# Autodesk Inventor assembly: 付け根_6_1
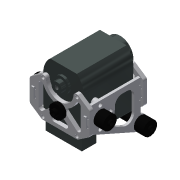
[picture p0: Inventor's stored thumbnail of the model, 180x180]
Saved by Autodesk Inventor 2016 (Build 200138000, 138)
## iProperties
Created: 2016-08-23
Part Number: 付け根_6_1
Material: 一般
Document SubType Name: Assembly
Designer: hiro
Mass: 143.306 g
Surface Area: 289.442 cm^2
Volume: 70.4906 cm^3
Density: 2.03298 g/cm^3
Author: hiro
## Documents named in this file (17)
- C:\Users\haya\Desktop\OpenPlatform\下半身_160823\付け根\付け根_6_1.iam
- C:\Users\haya\Desktop\OpenPlatform\既製品\B3M11xx.ipt
- B3M11xx.ipt
- C:\Users\haya\Desktop\OpenPlatform\下半身_160823\付け根\付け根_メインフレーム_6_1.ipt
- C:\Users\haya\Desktop\OpenPlatform\下半身_160823\付け根\付け根_サブフレーム_6_1.ipt
- C:\Users\haya\Desktop\OpenPlatform\下半身_160823\膝\膝_サブフレーム_6_4.ipt
- C:\Users\haya\Desktop\OpenPlatform\既製品\新規購入\AMP-340E.ipt
- C:\Users\haya\Desktop\OpenPlatform\既製品\新規購入\D3040-7815B.ipt
- C:\Users\haya\Desktop\OpenPlatform\既製品\新規購入\D3040-7115B.ipt
- C:\Users\haya\Desktop\OpenPlatform\既製品\新規購入\BRU-306_5.ipt
- C:\Users\haya\Desktop\OpenPlatform\下半身_160823\追加工\付け根_フリー軸_1_1_ver追加工.ipt
- C:\Users\haya\Desktop\OpenPlatform\既製品\新規購入\LL-7211-10.ipt
- C:\Users\haya\Desktop\OpenPlatform\既製品\新規購入\LL-7211-08.ipt
- C:\Users\haya\Desktop\OpenPlatform\下半身\付け根\付け根_サブフレーム_1_4.ipt
- C:\Users\haya\Desktop\OpenPlatform\既製品\CC-0311-08B.ipt
- C:\Users\haya\Desktop\OpenPlatform\下半身_160823\付け根\付け根_サブフレーム_6_2.ipt
- C:\Users\haya\Desktop\OpenPlatform\既製品\新規購入\BRU-305_5.ipt
## Components (30 placed, 15 different names)
1. B3M11xx:1 — メイト:1, メイト:2, メイト:3, 挿入:9, 挿入:10, 挿入:11, 挿入:12, 挿入:13, 挿入:14, 挿入:15, 挿入:16
2. 付け根_メインフレーム_6_1:1 — 挿入:13, 挿入:14, 挿入:15, 挿入:16, メイト:8, メイト:9, メイト:10, メイト:11, メイト:12, メイト:13, 挿入:60, 挿入:62
3. 付け根_サブフレーム_6_1:1 — メイト:7, メイト:10, メイト:11, メイト:13, 挿入:29, 角度:1, 挿入:31, 挿入:36, 挿入:39, 挿入:40, 挿入:41, 挿入:49
4. 付け根_サブフレーム_6_1:2 — メイト:7, メイト:8, メイト:9, メイト:12, 挿入:30, メイト:14, メイト:15, 挿入:42, 挿入:43, 挿入:44, 挿入:50
5. 付け根_メインフレーム_6_1:2 — 挿入:9, 挿入:10, 挿入:11, 挿入:12, 挿入:58
6. AMP-340E:1 — 挿入:29, 角度:1, 挿入:30
7. D3040-7815B:1 — 挿入:65, 挿入:70
8. D3040-7115B:1 — 挿入:45, 挿入:68
9. BRU-306_5:1 — 挿入:31, 挿入:70
10. BRU-306_5:2 — 挿入:37, 挿入:68
11. 膝_サブフレーム_6_4:1 — メイト:14, メイト:15, 挿入:37
12. 膝_サブフレーム_6_4:2 — 挿入:36
13. 付け根_フリー軸_1_1_ver追加工:1 — 挿入:42, 挿入:43, 挿入:44
14. 付け根_フリー軸_1_1_ver追加工:2 — 挿入:39, 挿入:40, 挿入:41
15. LL-7211-10:1 — 挿入:45
16. LL-7211-08:1 — 挿入:65
17. LL-7211-08:2 — 挿入:54
18. LL-7211-10:2 — 挿入:52
19. D3040-7815B:2 — 挿入:54, 挿入:69
20. D3040-7115B:2 — 挿入:52, 挿入:67
21. BRU-306_5:3 — 挿入:50, 挿入:64, 挿入:67
22. BRU-306_5:4 — 挿入:49, 挿入:66, 挿入:69
23. 膝_サブフレーム_6_4:3 — 挿入:66
24. 膝_サブフレーム_6_4:4 — 挿入:64
25. 付け根_サブフレーム_1_4:1 — 挿入:57
26. CC-0311-08B:1 — 挿入:57, 挿入:58
27. LL-7211-10:3 — 挿入:59
28. D3040-7115B:3 — 挿入:59, 挿入:61, 挿入:63
29. 付け根_サブフレーム_6_2:1 — 挿入:60, 挿入:61
30. BRU-305_5:1 — 挿入:62, 挿入:63
## Relationships (51: Insert 38, Mate 12, Angle 1)
- メイト:1 [Mate] (-19.75 mm): B3M11xx:1
- メイト:2 [Mate] (-25.75 mm): B3M11xx:1
- メイト:3 [Mate] (-16 mm): B3M11xx:1
- メイト:7 [Mate]: 付け根_サブフレーム_6_1:1 ↔ 付け根_サブフレーム_6_1:2
- 挿入:9 [Insert]: B3M11xx:1 ↔ 付け根_メインフレーム_6_1:2
- 挿入:10 [Insert]: B3M11xx:1 ↔ 付け根_メインフレーム_6_1:2
- 挿入:11 [Insert]: B3M11xx:1 ↔ 付け根_メインフレーム_6_1:2
- 挿入:12 [Insert]: B3M11xx:1 ↔ 付け根_メインフレーム_6_1:2
- 挿入:13 [Insert]: B3M11xx:1 ↔ 付け根_メインフレーム_6_1:1
- 挿入:14 [Insert]: B3M11xx:1 ↔ 付け根_メインフレーム_6_1:1
- 挿入:15 [Insert]: B3M11xx:1 ↔ 付け根_メインフレーム_6_1:1
- 挿入:16 [Insert]: B3M11xx:1 ↔ 付け根_メインフレーム_6_1:1
- メイト:8 [Mate] (0.005 mm): 付け根_メインフレーム_6_1:1 ↔ 付け根_サブフレーム_6_1:2
- メイト:9 [Mate] (0.005 mm): 付け根_メインフレーム_6_1:1 ↔ 付け根_サブフレーム_6_1:2
- メイト:10 [Mate] (0.005 mm): 付け根_メインフレーム_6_1:1 ↔ 付け根_サブフレーム_6_1:1
- メイト:11 [Mate] (0.005 mm): 付け根_メインフレーム_6_1:1 ↔ 付け根_サブフレーム_6_1:1
- メイト:12 [Mate]: 付け根_メインフレーム_6_1:1 ↔ 付け根_サブフレーム_6_1:2
- メイト:13 [Mate]: 付け根_メインフレーム_6_1:1 ↔ 付け根_サブフレーム_6_1:1
- 挿入:29 [Insert]: 付け根_サブフレーム_6_1:1 ↔ AMP-340E:1
- 角度:1 [Angle] (0 deg): 付け根_サブフレーム_6_1:1 ↔ AMP-340E:1
- 挿入:30 [Insert]: 付け根_サブフレーム_6_1:2 ↔ AMP-340E:1
- 挿入:31 [Insert]: 付け根_サブフレーム_6_1:1 ↔ BRU-306_5:1
- 挿入:36 [Insert]: 付け根_サブフレーム_6_1:1 ↔ 膝_サブフレーム_6_4:2
- メイト:14 [Mate]: 付け根_サブフレーム_6_1:2 ↔ 膝_サブフレーム_6_4:1
- メイト:15 [Mate]: 付け根_サブフレーム_6_1:2 ↔ 膝_サブフレーム_6_4:1
- 挿入:37 [Insert]: BRU-306_5:2 ↔ 膝_サブフレーム_6_4:1
- 挿入:39 [Insert]: 付け根_サブフレーム_6_1:1 ↔ 付け根_フリー軸_1_1_ver追加工:2
- 挿入:40 [Insert]: 付け根_サブフレーム_6_1:1 ↔ 付け根_フリー軸_1_1_ver追加工:2
- 挿入:41 [Insert]: 付け根_サブフレーム_6_1:1 ↔ 付け根_フリー軸_1_1_ver追加工:2
- 挿入:42 [Insert]: 付け根_サブフレーム_6_1:2 ↔ 付け根_フリー軸_1_1_ver追加工:1
- 挿入:43 [Insert]: 付け根_サブフレーム_6_1:2 ↔ 付け根_フリー軸_1_1_ver追加工:1
- 挿入:44 [Insert]: 付け根_サブフレーム_6_1:2 ↔ 付け根_フリー軸_1_1_ver追加工:1
- 挿入:45 [Insert]: D3040-7115B:1 ↔ LL-7211-10:1
- 挿入:49 [Insert]: 付け根_サブフレーム_6_1:1 ↔ BRU-306_5:4
- 挿入:50 [Insert]: 付け根_サブフレーム_6_1:2 ↔ BRU-306_5:3
- 挿入:52 [Insert]: LL-7211-10:2 ↔ D3040-7115B:2
- 挿入:54 [Insert]: LL-7211-08:2 ↔ D3040-7815B:2
- 挿入:57 [Insert]: 付け根_サブフレーム_1_4:1 ↔ CC-0311-08B:1
- 挿入:58 [Insert]: 付け根_メインフレーム_6_1:2 ↔ CC-0311-08B:1
- 挿入:59 [Insert]: LL-7211-10:3 ↔ D3040-7115B:3
- 挿入:60 [Insert]: 付け根_メインフレーム_6_1:1 ↔ 付け根_サブフレーム_6_2:1
- 挿入:61 [Insert]: D3040-7115B:3 ↔ 付け根_サブフレーム_6_2:1
- 挿入:62 [Insert]: 付け根_メインフレーム_6_1:1 ↔ BRU-305_5:1
- 挿入:63 [Insert]: D3040-7115B:3 ↔ BRU-305_5:1
- 挿入:64 [Insert]: BRU-306_5:3 ↔ 膝_サブフレーム_6_4:4
- 挿入:65 [Insert]: D3040-7815B:1 ↔ LL-7211-08:1
- 挿入:66 [Insert]: BRU-306_5:4 ↔ 膝_サブフレーム_6_4:3
- 挿入:67 [Insert]: D3040-7115B:2 ↔ BRU-306_5:3
- 挿入:68 [Insert]: D3040-7115B:1 ↔ BRU-306_5:2
- 挿入:69 [Insert]: D3040-7815B:2 ↔ BRU-306_5:4
- 挿入:70 [Insert]: D3040-7815B:1 ↔ BRU-306_5:1
